# Autodesk Inventor assembly: Chassis with place holders
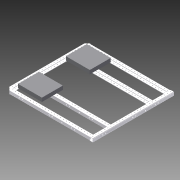
[picture p0: Inventor's stored thumbnail of the model, 180x180]
Saved by Autodesk Inventor 2014 SP1 (Build 180222100, 222)
## iProperties
Created: 2014-01-15
Part Number: Chassis with place holders
Document SubType Name: Assembly
Designer: Pradhan Alexander
Author: Pradhan Alexander
## Documents named in this file (9)
- K:\MHS\Technology\Holliday B\Group Projects\Robotics\CAD Team\CAD Team 2014\Chassis 2014\Chassis with place holders.iam
- K:\MHS\Technology\Holliday B\Group Projects\Robotics\CAD Team\CAD Team 2014\Chassis 2014\Chassis_Channel_AndyMark_am-0202-27in.ipt
- K:\MHS\Technology\Holliday B\Group Projects\Robotics\CAD Team\CAD Team 2014\Chassis 2014\Chassis_Channel_AndyMark_am-0202-27in-45.ipt
- K:\MHS\Technology\Holliday B\Group Projects\Robotics\CAD Team\CAD Team 2014\Chassis 2014\Chassis_Channel_AndyMark_am-0202-26.875.ipt
- K:\MHS\Technology\Holliday B\Group Projects\Robotics\CAD Team\CAD Team 2014\Chassis 2014\Toughbox-mini with long shaft.iam
- K:\MHS\Technology\Holliday B\Group Projects\Robotics\CAD Team\CAD Team 2014\Chassis 2014\8-mecanum-right-with-roller with hub.iam
- K:\MHS\Technology\Holliday B\Group Projects\Robotics\CAD Team\CAD Team 2014\Chassis 2014\8-mecanum-left-with-roller with hub.iam
- K:\MHS\Technology\Holliday B\Group Projects\Robotics\CAD Team\CAD Team 2014\shooter\Imported Components\top_level_ri3d\PIVOT_FRAMING.iam
- K:\MHS\Technology\Holliday B\Group Projects\Robotics\CAD Team\CAD Team 2014\Chassis 2014\Place holder for wheels.ipt
## Components (17 placed, 8 different names)
1. Chassis_Channel_AndyMark_am-0202-27in:2 — Mate:8, Flush:14, Flush:15, Flush:20, Flush:21
2. Chassis_Channel_AndyMark_am-0202-27in-45:1 — Mate:1, Flush:1, Flush:2, Mate:6, Flush:7, Mate:7, Flush:9, Mate:11, Angle:2, Mate:13, Angle:3, Mate:17, Flush:18, Flush:19, Flush:22, Flush:25
3. Chassis_Channel_AndyMark_am-0202-26.875:1 — Mate:7, Flush:9, Mate:9, Mate:18, Mate:21, Mate:27, Mate:28
4. Chassis_Channel_AndyMark_am-0202-26.875:2 — Mate:17, Flush:18, Flush:19, Flush:20, Flush:21, Flush:23
5. Chassis_Channel_AndyMark_am-0202-26.875:3 — Mate:1, Flush:1, Flush:2, Mate:8, Flush:14, Flush:15, Flush:24
6. Chassis_Channel_AndyMark_am-0202-26.875:4 — Mate:6, Flush:7, Mate:14, Angle:4, Mate:22, Mate:23, Mate:26
7. Toughbox-mini with long shaft:3 [sub-assembly] — Mate:18, Mate:19
8. 8-mecanum-right-with-roller with hub:2 [sub-assembly] — Mate:19
9. 8-mecanum-left-with-roller with hub:1 [sub-assembly] — Mate:24
10. Toughbox-mini with long shaft:4 [sub-assembly] — Mate:21
11. 8-mecanum-right-with-roller with hub:3 [sub-assembly]
12. Toughbox-mini with long shaft:5 [sub-assembly] — Mate:22, Mate:24
13. 8-mecanum-left-with-roller with hub:2 [sub-assembly] — Mate:25
14. Toughbox-mini with long shaft:6 [sub-assembly] — Mate:23, Mate:25
15. PIVOT_FRAMING:1 [sub-assembly] — Mate:28
16. Place holder for wheels:1 — Mate:26, Flush:22, Flush:23
17. Place holder for wheels:2 — Mate:27, Flush:24, Flush:25
## Relationships (43: Mate 24, Flush 16, Angle 3)
- Mate:1: Chassis_Channel_AndyMark_am-0202-27in-45:1 ↔ Chassis_Channel_AndyMark_am-0202-26.875:3
- Flush:1: Chassis_Channel_AndyMark_am-0202-27in-45:1 ↔ Chassis_Channel_AndyMark_am-0202-26.875:3
- Flush:2: Chassis_Channel_AndyMark_am-0202-27in-45:1 ↔ Chassis_Channel_AndyMark_am-0202-26.875:3
- Mate:6: Chassis_Channel_AndyMark_am-0202-27in-45:1 ↔ Chassis_Channel_AndyMark_am-0202-26.875:4
- Flush:7: Chassis_Channel_AndyMark_am-0202-27in-45:1 ↔ Chassis_Channel_AndyMark_am-0202-26.875:4
- Mate:7: Chassis_Channel_AndyMark_am-0202-27in-45:1 ↔ Chassis_Channel_AndyMark_am-0202-26.875:1
- Flush:9: Chassis_Channel_AndyMark_am-0202-27in-45:1 ↔ Chassis_Channel_AndyMark_am-0202-26.875:1
- Mate:8: Chassis_Channel_AndyMark_am-0202-27in:2 ↔ Chassis_Channel_AndyMark_am-0202-26.875:3
- Flush:14: Chassis_Channel_AndyMark_am-0202-27in:2 ↔ Chassis_Channel_AndyMark_am-0202-26.875:3
- Flush:15: Chassis_Channel_AndyMark_am-0202-27in:2 ↔ Chassis_Channel_AndyMark_am-0202-26.875:3
- Mate:9: Chassis_Channel_AndyMark_am-0202-26.875:1
- Mate:10
- Mate:11: Chassis_Channel_AndyMark_am-0202-27in-45:1
- Mate:12
- Angle:2 (90 deg): Chassis_Channel_AndyMark_am-0202-27in-45:1
- Flush:16
- Mate:13: Chassis_Channel_AndyMark_am-0202-27in-45:1
- Mate:14: Chassis_Channel_AndyMark_am-0202-26.875:4
- Mate:15
- Angle:3 (90 deg): Chassis_Channel_AndyMark_am-0202-27in-45:1
- Mate:16
- Angle:4 (0 deg): Chassis_Channel_AndyMark_am-0202-26.875:4
- Flush:17
- Mate:17: Chassis_Channel_AndyMark_am-0202-27in-45:1 ↔ Chassis_Channel_AndyMark_am-0202-26.875:2
- Flush:18: Chassis_Channel_AndyMark_am-0202-27in-45:1 ↔ Chassis_Channel_AndyMark_am-0202-26.875:2
- Flush:19: Chassis_Channel_AndyMark_am-0202-27in-45:1 ↔ Chassis_Channel_AndyMark_am-0202-26.875:2
- Flush:20: Chassis_Channel_AndyMark_am-0202-27in:2 ↔ Chassis_Channel_AndyMark_am-0202-26.875:2
- Flush:21: Chassis_Channel_AndyMark_am-0202-27in:2 ↔ Chassis_Channel_AndyMark_am-0202-26.875:2
- Mate:18: Chassis_Channel_AndyMark_am-0202-26.875:1 ↔ Toughbox-mini with long shaft:3
- Mate:19: Toughbox-mini with long shaft:3 ↔ 8-mecanum-right-with-roller with hub:2
- [Mate]: Toughbox-mini with long shaft:4 ↔ 8-mecanum-right-with-roller with hub:3
- Mate:21: Chassis_Channel_AndyMark_am-0202-26.875:1 ↔ Toughbox-mini with long shaft:4
- Mate:22: Chassis_Channel_AndyMark_am-0202-26.875:4 ↔ Toughbox-mini with long shaft:5
- Mate:23: Chassis_Channel_AndyMark_am-0202-26.875:4 ↔ Toughbox-mini with long shaft:6
- Mate:24: 8-mecanum-left-with-roller with hub:1 ↔ Toughbox-mini with long shaft:5
- Mate:25: 8-mecanum-left-with-roller with hub:2 ↔ Toughbox-mini with long shaft:6
- Mate:26: Chassis_Channel_AndyMark_am-0202-26.875:4 ↔ Place holder for wheels:1
- Flush:22 (50.8 mm): Chassis_Channel_AndyMark_am-0202-27in-45:1 ↔ Place holder for wheels:1
- Flush:23 (50.8 mm): Chassis_Channel_AndyMark_am-0202-26.875:2 ↔ Place holder for wheels:1
- Mate:27: Chassis_Channel_AndyMark_am-0202-26.875:1 ↔ Place holder for wheels:2
- Flush:24 (50.8 mm): Chassis_Channel_AndyMark_am-0202-26.875:3 ↔ Place holder for wheels:2
- Flush:25 (50.8 mm): Chassis_Channel_AndyMark_am-0202-27in-45:1 ↔ Place holder for wheels:2
- Mate:28: Chassis_Channel_AndyMark_am-0202-26.875:1 ↔ PIVOT_FRAMING:1
## Named parameters: d51_d50 = 0 mm
